# Autodesk Inventor assembly: ASSEMBLY_Part_Detector
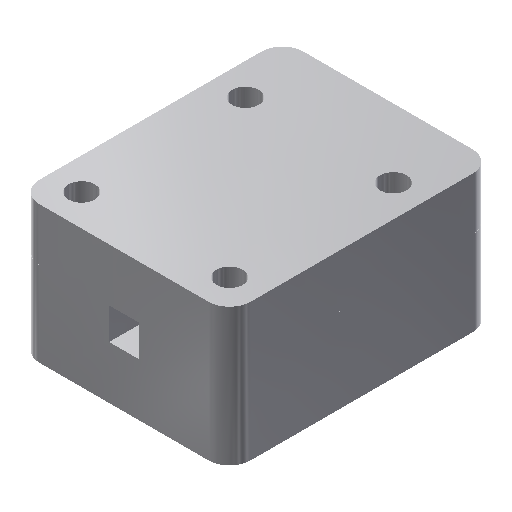
[picture p0: Inventor's stored thumbnail of the model, 512x512]
Saved by Autodesk Inventor 2025 (Build 290162010, 162A)
## iProperties
Created: 2018-07-20
Part Number: ASSEMBLY_Part_Detector
Document SubType Name: Assembly
Designer: Andrzej
Author: Andrzej
## Documents named in this file (4)
- D:\_ANDRZEJ_LACZEWSKI\_OTHER\MLTDIS - Measurement rail for SMD parts\MCAD\1_REV1\ASSEMBLY_MAIN_REVA\ASSEMBLY_Part_Detector.iam
- D:\_ANDRZEJ_LACZEWSKI\_OTHER\MLTDIS - Measurement rail for SMD parts\MCAD\1_REV1\ASSEMBLY_MAIN_REVA\3DP_PLA_Part_Detector_Bottom_Half.ipt
- D:\_ANDRZEJ_LACZEWSKI\_OTHER\MLTDIS - Measurement rail for SMD parts\MCAD\1_REV1\__COTS_PARTS\COTS_Vishay_TCST1230_Optocoupler.ipt
- D:\_ANDRZEJ_LACZEWSKI\_OTHER\MLTDIS - Measurement rail for SMD parts\MCAD\1_REV1\ASSEMBLY_MAIN_REVA\3DP_PLA_Part_Detector_Top_Half.ipt
## Components (3 placed, 3 different names)
1. 3DP_PLA_Part_Detector_Bottom_Half:1 — Mate:2, Mate:3, Mate:4, Mate:5, Flush:1, Flush:2
2. COTS_Vishay_TCST1230_Optocoupler:1 — Mate:2, Mate:3, Mate:4
3. 3DP_PLA_Part_Detector_Top_Half:1 — Mate:5, Flush:1, Flush:2
## Relationships (6: Mate 4, Flush 2)
- Mate:2: 3DP_PLA_Part_Detector_Bottom_Half:1 ↔ COTS_Vishay_TCST1230_Optocoupler:1
- Mate:3: 3DP_PLA_Part_Detector_Bottom_Half:1 ↔ COTS_Vishay_TCST1230_Optocoupler:1
- Mate:4: 3DP_PLA_Part_Detector_Bottom_Half:1 ↔ COTS_Vishay_TCST1230_Optocoupler:1
- Mate:5: 3DP_PLA_Part_Detector_Bottom_Half:1 ↔ 3DP_PLA_Part_Detector_Top_Half:1
- Flush:1: 3DP_PLA_Part_Detector_Bottom_Half:1 ↔ 3DP_PLA_Part_Detector_Top_Half:1
- Flush:2: 3DP_PLA_Part_Detector_Bottom_Half:1 ↔ 3DP_PLA_Part_Detector_Top_Half:1
